# Autodesk Inventor assembly: MotorMount
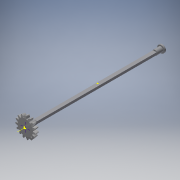
[picture p0: Inventor's stored thumbnail of the model, 180x180]
Saved by Autodesk Inventor 2017 (Build 210142000, 142)
## iProperties
Created: 2017-01-13
Part Number: MotorMount
Document SubType Name: Assembly
Designer: David Kopala
Author: David Kopala
## Documents named in this file (3)
- Z:\Documents\Drone\Drone\3D Models\Project\Chasis_03\MotorMount.iam
- Z:\Documents\Drone\Drone\3D Models\Project\Chasis_03\MotorMount_Part.ipt
- Z:\Documents\Drone\Drone\3D Models\Project\Chasis_03\Bevel_Inner_Reference\Design Accelerator\Bevel Gear21.ipt
## Components (2 placed, 2 different names)
1. MotorMount_Part:1 — Mate:1, Insert:1
2. Bevel Gear2:1 — Mate:1, Insert:1
## Relationships (2: Mate 1, Insert 1)
- Mate:1: MotorMount_Part:1 ↔ Bevel Gear2:1
- Insert:1: MotorMount_Part:1 ↔ Bevel Gear2:1
